# Autodesk Inventor assembly: prednji deo assembly
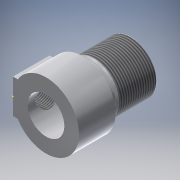
[picture p0: Inventor's stored thumbnail of the model, 180x180]
Saved by Autodesk Inventor 2019 (Build 230136000, 136)
## iProperties
Created: 2018-11-25
Part Number: prednji deo assembly
Document SubType Name: Assembly
Designer: aleks
Author: aleks
## Documents named in this file (3)
- C:\Users\aleks\OneDrive\Desktop\novi klip\prednji deo assembly.iam
- C:\Users\aleks\OneDrive\Desktop\novi klip\ulozak prednji.ipt
- C:\Users\aleks\OneDrive\Desktop\novi klip\prednji deo.ipt
## Components (2 placed, 2 different names)
1. prednji deo:1 — Mate:1
2. ulozak prednji:1 — Mate:1
## Relationships (1: Mate 1)
- Mate:1: prednji deo:1 ↔ ulozak prednji:1
